# Autodesk Inventor assembly: Full
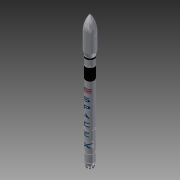
[picture p0: Inventor's stored thumbnail of the model, 180x180]
Saved by Autodesk Inventor 2015 (Build 190159000, 159)
## iProperties
Created: 2015-07-28
Part Number: Full
Document SubType Name: Assembly
Designer: Kevin
Author: Kevin
## Documents named in this file (4)
- E:\Documents\Inventor\Rocket\Full.iam
- E:\Documents\Inventor\Rocket\Body new.ipt
- E:\Documents\Inventor\Rocket\Engine 1.ipt
- E:\Documents\Inventor\Rocket\Head.ipt
## Components (11 placed, 3 different names)
1. Body new:1 — Mate:1, Mate:2, Mate:3, Mate:4, Mate:5, Mate:6, Mate:7, Mate:8, Mate:9, Mate:10, Mate:11, Mate:12, Mate:13, Mate:14, Mate:15, Mate:16, Mate:17, Mate:18, Mate:19, Mate:20, Mate:21
2. Engine 1:1 — Mate:9, Mate:10
3. Engine 1:2 — Mate:11, Mate:12
4. Engine 1:3 — Mate:7, Mate:8
5. Engine 1:4 — Mate:3, Mate:4
6. Engine 1:5 — Mate:1, Mate:2
7. Engine 1:6 — Mate:5, Mate:6
8. Engine 1:7 — Mate:13, Mate:14
9. Engine 1:8 — Mate:15, Mate:16
10. Engine 1:9 — Mate:17, Mate:18
11. Head:1 — Mate:19, Mate:20, Mate:21
## Relationships (21: Mate 21)
- Mate:1: Body new:1 ↔ Engine 1:5
- Mate:2: Body new:1 ↔ Engine 1:5
- Mate:3: Body new:1 ↔ Engine 1:4
- Mate:4: Body new:1 ↔ Engine 1:4
- Mate:5: Body new:1 ↔ Engine 1:6
- Mate:6: Body new:1 ↔ Engine 1:6
- Mate:7: Body new:1 ↔ Engine 1:3
- Mate:8: Body new:1 ↔ Engine 1:3
- Mate:9: Body new:1 ↔ Engine 1:1
- Mate:10: Body new:1 ↔ Engine 1:1
- Mate:11: Body new:1 ↔ Engine 1:2
- Mate:12: Body new:1 ↔ Engine 1:2
- Mate:13: Body new:1 ↔ Engine 1:7
- Mate:14: Body new:1 ↔ Engine 1:7
- Mate:15: Body new:1 ↔ Engine 1:8
- Mate:16: Body new:1 ↔ Engine 1:8
- Mate:17: Body new:1 ↔ Engine 1:9
- Mate:18 (2.032 mm): Body new:1 ↔ Engine 1:9
- Mate:19: Body new:1 ↔ Head:1
- Mate:20: Body new:1 ↔ Head:1
- Mate:21: Body new:1 ↔ Head:1
